# Autodesk Inventor assembly: Motor Assembly
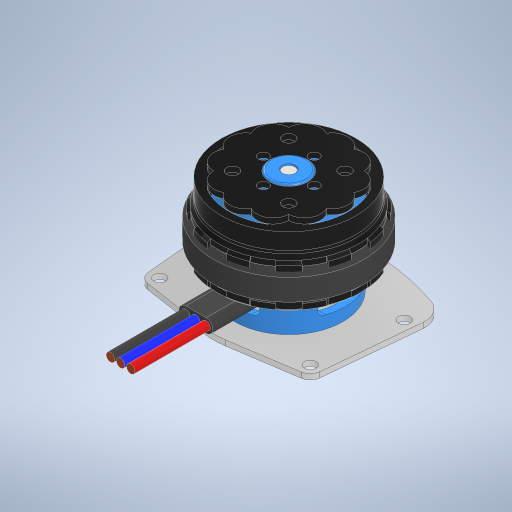
[picture p0: Inventor's stored thumbnail of the model, 512x512]
Saved by Autodesk Inventor 2023.2 (Build 272271000, 271)
## iProperties
Created: 2022-12-29
Part Number: Motor Assembly
Document SubType Name: Assembly
Designer: Nathan Cai
Mass: 110.978 g
Surface Area: 283.561 cm^2
Volume: 23.3648 cm^3
Density: 4.74978 g/cm^3
Author: Nathan Cai
## Documents named in this file (6)
- C:\Users\Nathan Cai\Documents\Inventor\Moon Cake V0.16\Motor Assembly.iam
- C:\Users\Nathan Cai\Documents\Inventor\Moon Cake V0.16\Motor Cap.ipt
- C:\Users\Nathan Cai\Documents\Inventor\Moon Cake V0.16\Motor Hub.ipt
- C:\Users\Nathan Cai\Documents\Inventor\Moon Cake V0.16\Motor Clutch.ipt
- C:\Users\Nathan Cai\Documents\Inventor\Moon Cake V0.16\Motor Plate.ipt
- C:\Users\Nathan Cai\Documents\Inventor\Moon Cake V0.16\Hobbyhh D3530 910KV\Hobbyhh D3530 910KV.iam
## Components (5 placed, 5 different names)
1. Motor Cap:1 — Mate:18, Mate:19, Mate:20, Mate:21
2. Motor Hub:1 — Mate:5, Mate:6, Mate:17, Mate:20
3. Motor Clutch:1 — Mate:5, Mate:6, Mate:13
4. Motor Plate:1 — Mate:13, Mate:14, Mate:15, Mate:16
5. Hobbyhh D3530 910KV:1 [sub-assembly] — Mate:14, Mate:15, Mate:16, Mate:17, Mate:18, Mate:19, Mate:21
## Relationships (11: Mate 11)
- Mate:5: Motor Hub:1 ↔ Motor Clutch:1
- Mate:6: Motor Hub:1 ↔ Motor Clutch:1
- Mate:13 (11.1125 mm): Motor Clutch:1 ↔ Motor Plate:1
- Mate:14: Motor Plate:1 ↔ Hobbyhh D3530 910KV:1
- Mate:15: Motor Plate:1 ↔ Hobbyhh D3530 910KV:1
- Mate:16: Motor Plate:1 ↔ Hobbyhh D3530 910KV:1
- Mate:17: Motor Hub:1 ↔ Hobbyhh D3530 910KV:1
- Mate:18: Motor Cap:1 ↔ Hobbyhh D3530 910KV:1
- Mate:19: Motor Cap:1 ↔ Hobbyhh D3530 910KV:1
- Mate:20: Motor Cap:1 ↔ Motor Hub:1
- Mate:21: Motor Cap:1 ↔ Hobbyhh D3530 910KV:1
